# Autodesk Inventor assembly: vane_mirror_pattern
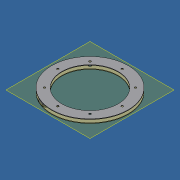
[picture p0: Inventor's stored thumbnail of the model, 180x180]
Saved by Autodesk Inventor 2022.4 (Build 264492010, 492A)
## iProperties
Created: 2006-08-01
Part Number: vane_mirror_pattern
Document SubType Name: Assembly
Designer: jmacmillan
Mass: 82.0722 g
Surface Area: 899.526 cm^2
Volume: 82.0722 cm^3
Density: 1 g/cm^3
CN_MASS: 0.08
Author: jmacmillan
## Documents named in this file (3)
- U:\Inventor 2022 Training\_Designer Training\Inventor 2022 - Advanced Assembly\Practice Files\Mirror and Pattern\vane_mirror_pattern.iam
- U:\Inventor 2022 Training\_Designer Training\Inventor 2022 - Advanced Assembly\Practice Files\Mirror and Pattern\Vane_Plate.ipt
- U:\Inventor 2022 Training\_Designer Training\Inventor 2022 - Advanced Assembly\Practice Files\Mirror and Pattern\Vane_blade.ipt
## Components (3 placed, 2 different names)
1. Vane_Plate:1 — Insert:1, Flush:1
2. Vane_blade:1 — Insert:1, Angle:1
3. Vane_Plate:2 — Mate:1
## Relationships (4: Insert 1, Angle 1, Flush 1, Mate 1)
- Insert:1: Vane_Plate:1 ↔ Vane_blade:1
- Angle:1 (0 deg): Vane_blade:1
- Flush:1 (4.5085 mm): Vane_Plate:1
- Mate:1 (4.5085 mm): Vane_Plate:2
